# Autodesk Inventor assembly: Capper Assembly
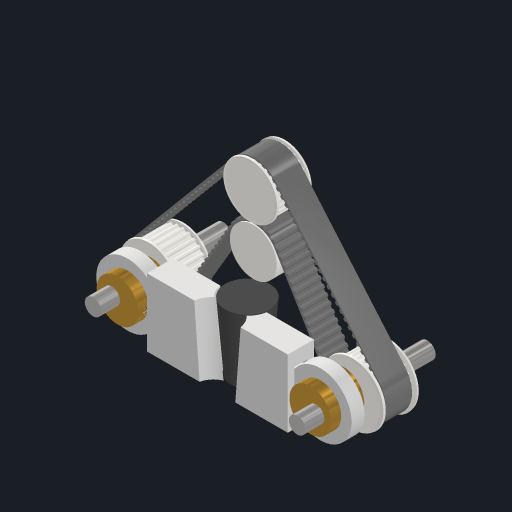
[picture p0: Inventor's stored thumbnail of the model, 512x512]
Saved by Autodesk Inventor 2023.1 (Build 271208000, 208)
## iProperties
Created: 2023-05-23
Part Number: Capper Assembly
Document SubType Name: Assembly
Designer: Jarrett
Author: Jarrett
## Documents named in this file (7)
- C:\Users\Jarrett\Desktop\Projects\BehrendURCMechanical\CAD\Science\Capper Assembly.iam
- C:\Users\Jarrett\Desktop\Projects\BehrendURCMechanical\CAD\Science\Capper Gate Bushing.ipt
- C:\Users\Jarrett\Desktop\Projects\BehrendURCMechanical\CAD\Science\Capper Gate Linkage.ipt
- C:\Users\Jarrett\Desktop\Projects\BehrendURCMechanical\CAD\Science\Capper Gate.ipt
- C:\Users\Jarrett\Desktop\Projects\BehrendURCMechanical\CAD\Science\Capper Gate Shaft.ipt
- C:\Users\Jarrett\Desktop\Projects\BehrendURCMechanical\CAD\Science\SC-1-01-Test Tube Cap.ipt
- C:\Users\Jarrett\Desktop\Projects\BehrendURCMechanical\CAD\Science\Capper Assembly\Design Accelerator\Synchronous Belts Transmission1.iam
## Components (10 placed, 6 different names)
1. Capper Gate Bushing:1 — Rotational:2, Flush:1, Mate:1, Mate:3, Mate:5
2. Capper Gate Linkage:1 — Rotational:2, Rotational:3
3. Capper Gate:1 — Mate:2, Rotational:3, Flush:3
4. Capper Gate Shaft:1 — Mate:3
5. SC-1-01-Test Tube Cap:1
6. Synchronous Belts Transmission:1 [sub-assembly]
7. Capper Gate Shaft:2 — Mate:6
8. Capper Gate Bushing:2 — Rotational:4, Flush:2, Mate:4, Mate:5, Mate:6
9. Capper Gate Linkage:2 — Rotational:4, Rotational:5
10. Capper Gate:2 — Rotational:5, Flush:3
## Relationships (13: Mate 6, RevoluteJoint 4, Flush 3)
- Rotational:2 [RevoluteJoint]: Capper Gate Bushing:1 ↔ Capper Gate Linkage:1
- Flush:1: Capper Gate Bushing:1
- Mate:1: Capper Gate Bushing:1
- Mate:2 (-13 mm): Capper Gate:1
- Rotational:3 [RevoluteJoint]: Capper Gate Linkage:1 ↔ Capper Gate:1
- Mate:3: Capper Gate Bushing:1 ↔ Capper Gate Shaft:1
- Rotational:4 [RevoluteJoint]: Capper Gate Bushing:2 ↔ Capper Gate Linkage:2
- Rotational:5 [RevoluteJoint]: Capper Gate Linkage:2 ↔ Capper Gate:2
- Flush:2: Capper Gate Bushing:2
- Flush:3: Capper Gate:1 ↔ Capper Gate:2
- Mate:4: Capper Gate Bushing:2
- Mate:5 (78.5 mm): Capper Gate Bushing:1 ↔ Capper Gate Bushing:2
- Mate:6: Capper Gate Shaft:2 ↔ Capper Gate Bushing:2
